# Autodesk Inventor assembly: Counter_Support_Ceramic
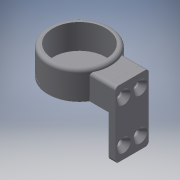
[picture p0: Inventor's stored thumbnail of the model, 180x180]
Saved by Autodesk Inventor 2017 (Build 210142000, 142)
## iProperties
Created: 2020-01-10
Part Number: Counter_Support_Ceramic
Document SubType Name: Assembly
Designer: Christian
Author: Christian
## Documents named in this file (3)
- E:\Work\Repos\personal\3d-design\02_Designs\01_home\counter support\counter_support..iam
- E:\Work\Repos\personal\3d-design\02_Designs\01_home\counter support\counter_support_b_base.ipt
- E:\Work\Repos\personal\3d-design\02_Designs\01_home\counter support\counter_support_b_leg.ipt
## Components (2 placed, 2 different names)
1. counter_support_b_base:1 — Flush:1, Flush:2
2. counter_support_b_leg:1 — Flush:1, Flush:2
## Relationships (2: Flush 2)
- Flush:1: counter_support_b_base:1 ↔ counter_support_b_leg:1
- Flush:2: counter_support_b_base:1 ↔ counter_support_b_leg:1
